# Autodesk Inventor assembly: GY81 Logger
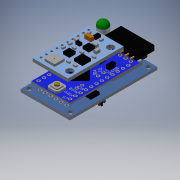
[picture p0: Inventor's stored thumbnail of the model, 180x180]
Saved by Autodesk Inventor 2016 (Build 200138000, 138)
## iProperties
Created: 2015-11-30
Part Number: GY81 Logger
Document SubType Name: Assembly
Designer: Spooner
Author: Spooner
## Documents named in this file (6)
- C:\Users\Spooner\Documents\GY81 Logger\3D Models\GY81 Logger.iam
- C:\Users\Spooner\Documents\GY81 Logger\3D Models\Arduino Pro Mini.ipt
- C:\Users\Spooner\Documents\GY81 Logger\3D Models\GY81.ipt
- C:\Users\Spooner\Documents\GY81 Logger\3D Models\MicroSD Card in Reader.iam
- C:\Users\Spooner\Documents\GY81 Logger\3D Models\Clipped LED.ipt
- C:\Users\Spooner\Documents\GY81 Logger\3D Models\Right-Angle Female Header.ipt
## Components (5 placed, 5 different names)
1. Arduino Pro Mini:1 — Flush:1, Flush:2, Mate:1, Mate:2, Mate:4, Mate:5, Mate:6
2. GY81:1 — Flush:3, Flush:4, Mate:2
3. MicroSD Card in Reader:1 [sub-assembly] — Flush:1, Flush:2, Mate:1, Flush:3, Flush:4, Mate:3, Flush:5, Flush:6
4. Clipped LED:1 — Mate:3, Flush:5, Flush:6
5. Right-Angle Female Header:1 — Mate:4, Mate:5, Mate:6
## Relationships (12: Flush 6, Mate 6)
- Flush:1: Arduino Pro Mini:1 ↔ MicroSD Card in Reader:1
- Flush:2: Arduino Pro Mini:1 ↔ MicroSD Card in Reader:1
- Mate:1 (5.08 mm): Arduino Pro Mini:1 ↔ MicroSD Card in Reader:1
- Flush:3: GY81:1 ↔ MicroSD Card in Reader:1
- Flush:4 (5.715 mm): GY81:1 ↔ MicroSD Card in Reader:1
- Mate:2 (2.54 mm): Arduino Pro Mini:1 ↔ GY81:1
- Mate:3 (3.81 mm): MicroSD Card in Reader:1 ↔ Clipped LED:1
- Flush:5 (3.81 mm): MicroSD Card in Reader:1 ↔ Clipped LED:1
- Flush:6 (3.175 mm): MicroSD Card in Reader:1 ↔ Clipped LED:1
- Mate:4: Arduino Pro Mini:1 ↔ Right-Angle Female Header:1
- Mate:5: Arduino Pro Mini:1 ↔ Right-Angle Female Header:1
- Mate:6: Arduino Pro Mini:1 ↔ Right-Angle Female Header:1
